# Autodesk Inventor assembly: Mesa
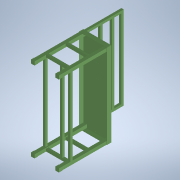
[picture p0: Inventor's stored thumbnail of the model, 180x180]
Saved by Autodesk Inventor 2021 (Build 250183000, 183)
## iProperties
Created: 2021-06-02
Part Number: Mesa
Document SubType Name: Assembly
Designer: Nelson
Author: Nelson
## Documents named in this file (8)
- D:\Nelson\Documentos\Inventor\PrensaHidraulica_Automatizada\Mesa.iam
- D:\Nelson\Documentos\Inventor\PrensaHidraulica_Automatizada\Mesa_tablero.ipt
- D:\Nelson\Documentos\Inventor\PrensaHidraulica_Automatizada\Mesa_pata.ipt
- D:\Nelson\Documentos\Inventor\PrensaHidraulica_Automatizada\Mesa_base1.ipt
- D:\Nelson\Documentos\Inventor\PrensaHidraulica_Automatizada\Mesa_base2.ipt
- D:\Nelson\Documentos\Inventor\PrensaHidraulica_Automatizada\Mesa_base3.ipt
- D:\Nelson\Documentos\Inventor\PrensaHidraulica_Automatizada\Mesa_soporte1.ipt
- D:\Nelson\Documentos\Inventor\PrensaHidraulica_Automatizada\Mesa_soporte2.ipt
## Components (17 placed, 7 different names)
1. Mesa_tablero:1 — Mate:1, Mate:2, Mate:3, Mate:4, Mate:5, Mate:6, Mate:7, Mate:8, Mate:9, Mate:10, Mate:11, Mate:12, Mate:24, Mate:25, Mate:26, Mate:27, Mate:28, Mate:29
2. Mesa_pata:1 — Mate:1, Mate:2, Mate:3, Mate:14, Flush:3
3. Mesa_pata:2 — Mate:4, Mate:5, Mate:6, Mate:13, Flush:2, Mate:15, Flush:5, Flush:6, Mate:19, Flush:10
4. Mesa_pata:3 — Mate:7, Mate:8, Mate:9, Flush:1, Flush:8, Mate:21, Flush:11
5. Mesa_pata:4 — Mate:10, Mate:11, Mate:12, Flush:4, Mate:16, Flush:7
6. Mesa_base1:1 — Mate:13, Flush:1, Flush:2, Mate:23
7. Mesa_base1:2 — Mate:14, Flush:3, Flush:4
8. Mesa_base2:1 — Mate:15, Flush:5, Flush:6, Mate:17, Flush:9, Mate:20
9. Mesa_base2:2 — Mate:16, Flush:7, Flush:8, Mate:22
10. Mesa_base3:1 — Mate:17, Flush:9, Mate:23
11. Mesa_base2:3 — Mate:19, Flush:10, Mate:20
12. Mesa_base2:4 — Mate:21, Flush:11, Mate:22
13. Mesa_soporte1:1 — Mate:24, Mate:25, Mate:26, Mate:30, Flush:12, Flush:13, Mate:31, Flush:14, Mate:32, Flush:16
14. Mesa_soporte1:2 — Mate:27, Mate:28, Mate:29
15. Mesa_soporte2:1 — Mate:30, Flush:12, Flush:13, Flush:15
16. Mesa_soporte2:2 — Mate:31, Flush:14, Flush:15, Mate:33
17. Mesa_soporte2:3 — Mate:32, Flush:16, Mate:33
## Relationships (48: Mate 32, Flush 16)
- Mate:1: Mesa_tablero:1 ↔ Mesa_pata:1
- Mate:2: Mesa_tablero:1 ↔ Mesa_pata:1
- Mate:3: Mesa_tablero:1 ↔ Mesa_pata:1
- Mate:4: Mesa_tablero:1 ↔ Mesa_pata:2
- Mate:5: Mesa_tablero:1 ↔ Mesa_pata:2
- Mate:6: Mesa_tablero:1 ↔ Mesa_pata:2
- Mate:7: Mesa_tablero:1 ↔ Mesa_pata:3
- Mate:8: Mesa_tablero:1 ↔ Mesa_pata:3
- Mate:9: Mesa_tablero:1 ↔ Mesa_pata:3
- Mate:10: Mesa_tablero:1 ↔ Mesa_pata:4
- Mate:11: Mesa_tablero:1 ↔ Mesa_pata:4
- Mate:12: Mesa_tablero:1 ↔ Mesa_pata:4
- Mate:13: Mesa_pata:2 ↔ Mesa_base1:1
- Flush:1: Mesa_pata:3 ↔ Mesa_base1:1
- Flush:2 (250 mm): Mesa_pata:2 ↔ Mesa_base1:1
- Mate:14: Mesa_pata:1 ↔ Mesa_base1:2
- Flush:3: Mesa_pata:1 ↔ Mesa_base1:2
- Flush:4 (250 mm): Mesa_pata:4 ↔ Mesa_base1:2
- Mate:15: Mesa_pata:2 ↔ Mesa_base2:1
- Flush:5: Mesa_pata:2 ↔ Mesa_base2:1
- Flush:6 (250 mm): Mesa_pata:2 ↔ Mesa_base2:1
- Mate:16: Mesa_pata:4 ↔ Mesa_base2:2
- Flush:7: Mesa_pata:4 ↔ Mesa_base2:2
- Flush:8 (250 mm): Mesa_pata:3 ↔ Mesa_base2:2
- Mate:17: Mesa_base2:1 ↔ Mesa_base3:1
- Flush:9: Mesa_base2:1 ↔ Mesa_base3:1
- Mate:19: Mesa_pata:2 ↔ Mesa_base2:3
- Flush:10: Mesa_pata:2 ↔ Mesa_base2:3
- Mate:20 (370 mm): Mesa_base2:1 ↔ Mesa_base2:3
- Mate:21: Mesa_pata:3 ↔ Mesa_base2:4
- Flush:11: Mesa_pata:3 ↔ Mesa_base2:4
- Mate:22 (370 mm): Mesa_base2:2 ↔ Mesa_base2:4
- Mate:23 (127 mm): Mesa_base1:1 ↔ Mesa_base3:1
- Mate:24: Mesa_tablero:1 ↔ Mesa_soporte1:1
- Mate:25: Mesa_tablero:1 ↔ Mesa_soporte1:1
- Mate:26: Mesa_tablero:1 ↔ Mesa_soporte1:1
- Mate:27: Mesa_tablero:1 ↔ Mesa_soporte1:2
- Mate:28: Mesa_tablero:1 ↔ Mesa_soporte1:2
- Mate:29: Mesa_tablero:1 ↔ Mesa_soporte1:2
- Mate:30: Mesa_soporte1:1 ↔ Mesa_soporte2:1
- Flush:12: Mesa_soporte1:1 ↔ Mesa_soporte2:1
- Flush:13: Mesa_soporte1:1 ↔ Mesa_soporte2:1
- Mate:31: Mesa_soporte1:1 ↔ Mesa_soporte2:2
- Flush:14: Mesa_soporte1:1 ↔ Mesa_soporte2:2
- Flush:15 (200 mm): Mesa_soporte2:1 ↔ Mesa_soporte2:2
- Mate:32: Mesa_soporte1:1 ↔ Mesa_soporte2:3
- Flush:16: Mesa_soporte1:1 ↔ Mesa_soporte2:3
- Mate:33 (200 mm): Mesa_soporte2:2 ↔ Mesa_soporte2:3
